# Autodesk Inventor assembly: Assembly13
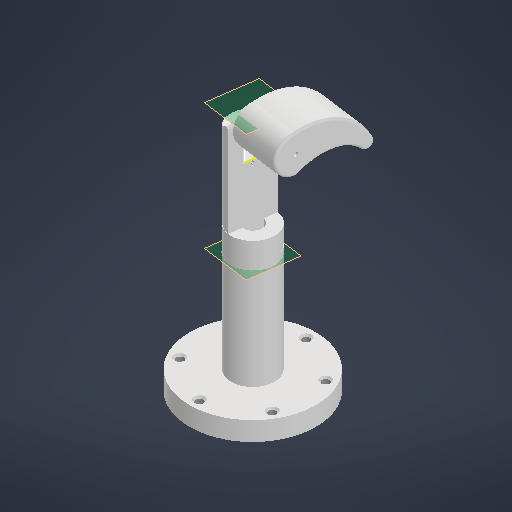
[picture p0: Inventor's stored thumbnail of the model, 512x512]
Saved by Autodesk Inventor 2026.2 (Build 302298000, 298)
## iProperties
Created: 2026-04-05
Part Number: Assembly13
Document SubType Name: Assembly
Designer: anasa
Author: anasa
## Documents named in this file (5)
- C:\Users\anasa\Desktop\Assembly13.iam
- C:\Users\anasa\Desktop\base.ipt
- C:\Users\anasa\Desktop\shaft.ipt
- C:\Users\anasa\Desktop\p1.ipt
- C:\Users\anasa\Desktop\p2.ipt
## Components (5 placed, 4 different names)
1. base:1 — Mate:1, Mate:2
2. shaft:1 — Mate:3, Mate:4, Mate:5
3. shaft:2 — Mate:1, Mate:2, Mate:5
4. p1:1 — Mate:3, Mate:4, Mate:6, Mate:7
5. p2:1 — Mate:6, Mate:7
## Relationships (7: Mate 7)
- Mate:1: base:1 ↔ shaft:2
- Mate:2: base:1 ↔ shaft:2
- Mate:3: shaft:1 ↔ p1:1
- Mate:4: shaft:1 ↔ p1:1
- Mate:5: shaft:1 ↔ shaft:2
- Mate:6: p1:1 ↔ p2:1
- Mate:7: p1:1 ↔ p2:1
